# Autodesk Inventor assembly: NSFMKRRA10-131-F3-S5-KA5-A19-KB111.5-B11
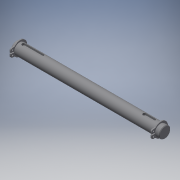
[picture p0: Inventor's stored thumbnail of the model, 180x180]
Saved by Autodesk Inventor 2019 (Build 230136000, 136)
## iProperties
Category: PARTsolutions
Company: MISUMI
Created: 2022-11-16
Part Number: NSFMKRRA10-131-F3-S5-KA5-A19-KB111.5-B11
Catalog Web Link: www.cadenas.de
Description: NSFMKRR, SFMKRR, PSFMKRR, SSFMKRR, NSFHKRR, SFHKRR, PSFHKRR, SSFHKRR, NSFGKRR, SFGKRR, PSFGKRR, SSFGKRR, NSFMKRRA, SFMKRRA, PSFMKRRA, SSFMKRRA, NSFHKRRA, SFHKRRA, PSFHKRRA, SSFHKRRA, NSFGKRRA, SFGKRRA, PSFGKRRA, SSFGKRRA-Rotary Shafts - Retaining Ring Grooves on Both Ends with Keyway -
Vendor: MISUMI
Document SubType Name: Assembly
Designer: psAdmin
Manufacturer: MISUMI
Mass: 10.2368 g
Surface Area: 47.8895 cm^2
Volume: 10.2368 cm^3
Density: 1 g/cm^3
Title: NSFMKRRA10-131-F3-S5-KA5-A19-KB111.5-B11
Author: Cadenas PARTsolutions
Comments: Rotary Shafts - Retaining Ring Grooves on Both Ends with Keyway -
PSOL_IDENT_0: {$CADENAS_DATA/23d-libs/misumi/metric/11_rotary_shafts/psfgkrr_asmtab.prj},644 {VTYP=3D},{STYP=ASSTA
PSOL_IDENT_1: B},{NB=NSFMKRRA10-131-F3-S5-KA5-A19-KB111.5-B11},{LINA=NSFMKRRA10-131-F3-S5-KA5-A19-KB111.5-B11},{NN=
PSOL_IDENT_2: NSFMKRR, SFMKRR, PSFMKRR, SSFMKRR, NSFHKRR, SFHKRR, PSFHKRR, SSFHKRR, NSFGKRR, SFGKRR, PSFGKRR, SSFG
PSOL_IDENT_3: KRR, NSFMKRRA, SFMKRRA, PSFMKRRA, SSFMKRRA, NSFHKRRA, SFHKRRA, PSFHKRRA, SSFHKRRA, NSFGKRRA, SFGKRRA
PSOL_IDENT_4: , PSFGKRRA, SSFGKRRA},{DATE=25.01.2022 23:09:58},{GEOMDATE=05.02.2021 08:16:43},{VERSION=},{LINEID=3
PSOL_IDENT_5: 0},{WBVAR=TS,TYS,MAT,ST,ALT1,L,F,S,NOK,KA,A,KB,B,KC,C,ALT3,FC,GALT3,WFC,J,WALT3,V,ALT4,SFC,SG,AG,ALT
PSOL_IDENT_6: 10,KWC,ALT11,WC,ALT5,UC,ALT7,SC,ALT32,CD},{WBNUMERIC=L,F,S,KA,A,KB,B,KC,C,FC,GALT3,WFC,J,WALT3,V,SFC
PSOL_IDENT_7: ,SG,AG,KWC,WC,UC,SC}  {NB=NSFMKRRA10-131-F3-S5-KA5-A19-KB111.5-B11},{LINA=NSFMKRRA10-131-F3-S5-KA5-A
PSOL_IDENT_8: 19-KB111.5-B11},{KT=DUMMY},{PN=NSFMKRRA10-131-F3-S5-KA5-A19-KB111.5-B11},{TS=A},{TSALG='','Standard'
PSOL_IDENT_9: ,'A','Retaining Ring'},{TYS=M},{TYSALG= 'M','h9 (Cold-drawn)','H','h7 (Ground)','G','g6 (Ground)' },
PSOL_IDENT_10: {MAT=S45C},{MATALG= 'S45C','S45C Equivalent', 'SUS304','304 Stainless Steel' },{ST=},{STALG= '','-','
PSOL_IDENT_11: BO','Black Oxide', 'ENP','Electroless Nickel Plating' },{TYPE=NSFMKRR},{D=10},{ALT1=},{LKCMAX=799.9}
PSOL_IDENT_12: ,{L=131.0},{LALG=[15:800/0.1]},{LMIN=15},{LMAX=800},{F=3.0},{FALG=[3:126/0.1]},{FMIN=3},{FMAX1=122.8
PSOL_IDENT_13: },{FMIN2=6.2},{FMAX2=126},{S=5.0},{SALG=[3:126/0.1]},{SMIN1=3},{SMAX1=121},{SMIN2=6.2},{SMAX2=126},{
PSOL_IDENT_14: DD=9.6},{MM=1.15},{MMALG=1.2},{MMJ=2},{NOK=2},{NOKALG= '1', 'with 1 Key Groove', '2'  , 'with 2 Key
PSOL_IDENT_15: Grooves', '3'  , 'with 3 Key Grooves'},{CIFNOK1=0},{CIFNOK2=3},{CIFNOK3=0},{TOL1=0},{TOL2=3},{TOL3=0
PSOL_IDENT_16: },{BB=3},{TT=1.8},{KA=5.0},{KAALG=[5:116/0.1]},{KAMIN1=0},{KAMIN2=5},{KAMIN3=129.2},{KAMAX1=-1000},{
PSOL_IDENT_17: KAMAX2=116},{KAMAX3=-1000},{A=19.0},{AALG=[3:100/0.1]},{AMIN=3},{AMAX=100},{AMAX1=-1000},{AMAX2=100}
PSOL_IDENT_18: ,{AMAX3=-1000},{KAPN=-KA5-A19},{KB=111.5},{KBALG=[26:121/0.1]},{KBMIN1=26},{KBMIN2=26},{KBMIN3=129.2
PSOL_IDENT_19: },{KBMAX1=-1000},{KBMAX2=121},{KBMAX3=-1000},{B=11.0},{BALG=[3:12.5/0.1]},{BMIN=3},{BMAX=12.5},{BMAX
PSOL_IDENT_20: 1=-1000},{BMAX2=12.5},{BMAX3=-1000},{KBPN=-KB111.5-B11},{KC=0.0},{KCALG=[0]},{KCMIN1=124.5},{KCMIN2=
PSOL_IDENT_21: 124.5},{KCMIN3=129.2},{KCMAX1=-1000},{KCMAX2=-1000},{KCMAX3=-1000},{C=0.0},{CALG=0},{CMIN=3},{CMAX=-
PSOL_IDENT_22: 1000},{CMAX1=-1000},{CMAX2=-1000},{CMAX3=-1000},{CIFKA=5},{CIFKB=3},{CIFKC=3},{KCPN=},{ALT3=},{ALT3A
PSOL_IDENT_23: LG= '', 'w/o Set Screw Flat','FC','with FC (Adds a Set Screw Flat)','WFC','with WFC (Adds Two Set Sc
PSOL_IDENT_24: rew Flats)','FCWFC','with FC + WFC (Adds Three Set Screw Flats)' },{ALT3PN=},{FC=0},{FCALG=[0]},{FCM
PSOL_IDENT_25: IN=0},{FCMAX=130},{GALT3=0},{GALT3ALG=[0]},{GALT3MIN=1},{GALT3MAX=70},{GALT3MAX2=70},{GALT3MAX3=70},
PSOL_IDENT_26: {WFC=0},{WFCALG=[0]},{WFCMIN=0},{WFCMIN2=2},{WFCMAX=127},{WFCMAX2=-3},{WFCMAX3=-4},{J=0},{JALG=[0]},
PSOL_IDENT_27: {JMIN=1},{JMAX=70},{JMAX2=-2},{JMAX3=-5},{WALT3=0},{WALT3ALG=[0]},{WALT3MIN=0},{WALT3MIN2=133},{WALT
PSOL_IDENT_28: 3MAX=128},{WALT3MAX2=128},{V=0},{VALG=[0]},{VMIN=1},{VMAX=70},{VMAX2=70},{CIFFC=0},{ALT4=},{ALT4ALG=
PSOL_IDENT_29: '', 'w/o SFC (2 Set Screw Flats (Angle Specified))', 'SFC'  , 'with SFC (2 Set Screw Flats (Angle S
PSOL_IDENT_30: pecified))'},{ALT4PN=},{SFC=0},{SFCALG=[0]},{SFCMIN=0},{SFCMAX=130},{SG=0},{SGALG=[0]},{SGMIN=1},{SG
PSOL_IDENT_31: MAX=70},{AG=0},{AGALG=[0]},{H=0},{CIFSFC=0},{ALT10=},{ALT10ALG= '','Not applicable' },{KWC=0},{KWCAL
PSOL_IDENT_32: G=[0]},{KWCMIN=1},{KWCMAX=0},{WALT10=8},{ALT10PN=},{ALT11=},{ALT11ALG= '','Not applicable' },{WC=0.0
PSOL_IDENT_33: },{WCALG=[0]},{ALT11PN=},{ALT5=},{ALT5ALG= '', 'w/o UC (Slit Cam Groove)', 'UC', 'with UC (Slit Cam
PSOL_IDENT_34: Groove)'},{ALT5PN=},{UC=0},{UCALG=[0]},{UCMIN=1},{UCMAX=125},{DDALT5=0},{LL1=0},{ALT7=},{ALT7ALG= ''
PSOL_IDENT_35: , 'w/o SC (Wrench Flats)', 'SC', 'with SC (Wrench Flats)'},{ALT7PN=},{SC=0},{SCALG=[0]},{SCMIN=0},{S
PSOL_IDENT_36: CMAX=123},{LL2=0},{LL2ALG=8},{WALT7=0},{CIFSC=0},{ALT32=},{ALT32ALG= '','w/o CD (Changes Part D Cham
PSOL_IDENT_37: fering)','CD','with CD (Changes Part D Chamfering)' },{CD=},{CDALG= '','N/A' },{CD3D=0.5},{ALT32PN=}
PSOL_IDENT_38: ,{CIF323R=0},{CIF323L=0},{CIF324R=0},{CIF324L=0},{CIF3210=0},{CIF32F=0},{CIF32S=0},{ERRORPN=},{ERROR
PSOL_IDENT_39: KGALT3=OK},{ERRORKGALT4=OK},{ERRORKGALT5=OK},{ERRORKGALT7=OK},{ERRORKGALT10=OK},{ERRORRALT3=OK},{ERR
PSOL_IDENT_40: ORRALT4=NG},{ERRORRALT5=NG},{ERRORRALT7=NG},{ERRORRALT10=OK},{ERRORALT34=OK},{ERRORALT35=OK},{ERRORA
PSOL_IDENT_41: LT37=OK},{ERRORALT310=OK},{ERRORALT45=OK},{ERRORALT47=OK},{ERRORALT410=OK},{ERRORALT57=OK},{ERRORALT
PSOL_IDENT_42: 510=OK},{ERRORALT710=OK},{PCUT3D=0},{QCUT3D=0},{TTALT2=1.8},{BBALT2=3},{PPATH=11_components/psfgkrr/
PSOL_IDENT_43: psfgkrr_asmtpl.prj}
NB: NSFMKRRA10-131-F3-S5-KA5-A19-KB111.5-B11
NN: NSFMKRR, SFMKRR, PSFMKRR, SSFMKRR, NSFHKRR, SFHKRR, PSFHKRR, SSFHKRR, NSFGKRR, SFGKRR, PSFGKRR, SSFGKRR, NSFMKRRA, SFMKRRA, PSFMKRRA, SSFMKRRA, NSFHKRRA, SFHKRRA, PSFHKRRA, SSFHKRRA, NSFGKRRA, SFGKRRA, PSFGKRRA, SSFGKRRA
NT: Rotary Shafts - Retaining Ring Grooves on Both Ends with Keyway -
NBSYN: $PN.
LINA: NSFMKRRA10-131-F3-S5-KA5-A19-KB111.5-B11
CATALOG: Misumi
PN: NSFMKRRA10-131-F3-S5-KA5-A19-KB111.5-B11
TS: Retaining Ring
TYS: h9 (Cold-drawn)
MAT: S45C Equivalent
ST: -
D: 10
ALT1: w/o LKC (Changes L Tolerance)
L: 131
F: 3
S: 5
DD: 9.6
MM: 1.15
NOK: with 2 Key Grooves
KA: 5
A: 19
KB: 111.5
B: 11
KC: 0
C: 0
ALT3: w/o Set Screw Flat
FC: 0
GALT3: 0
WFC: 0
J: 0
WALT3: 0
V: 0
ALT4: w/o SFC (2 Set Screw Flats (Angle Specified))
SFC: 0
SG: 0
AG: 0
H: 0
ALT10: Not applicable
KWC: 0
ALT11: Not applicable
WC: 0
ALT5: w/o UC (Slit Cam Groove)
UC: 0
DDALT5: 0
LL1: 0
ALT7: w/o SC (Wrench Flats)
SC: 0
LL2: 0
WALT7: 0
ALT32: w/o CD (Changes Part D Chamfering)
CD: N/A
SUPPLIER: MISUMI
ARTICLENO: NSFMKRRA10-131-F3-S5-KA5-A19-KB111.5-B11
BOMINFO: NSFMKRRA10-131-F3-S5-KA5-A19-KB111.5-B11
CREATOR: CADENAS GmbH
## Documents named in this file (3)
- e:\temp\worker_COMMON_4\temp\tmp_3352_176_HThwi\format_0\NSFMKRRA10-131-F3-S5-KA5-A19-KB111_5-B11.iam
- e:\temp\worker_COMMON_4\temp\tmp_3352_176_HThwi\format_0\NSFMKRRA10-131-F3-S5-KA5-A19-KB111_5-B11_s.ipt
- e:\temp\worker_COMMON_4\temp\tmp_3352_176_HThwi\format_0\STWS10.ipt
## Components (3 placed, 2 different names)
1. NSFMKRRA10-131-F3-S5-KA5-A19-KB111_5-B11_s:1 — to_rring_1_XY@1 <-> 1_XY@2, to_rring_1_Z@1 <-> 1_Z@2, to_rring_1_YZ@1 <-> 1_YZ@2, to_rring_2_XY@1 <-> 1_XY@3, to_rring_2_Z@1 <-> 1_Z@3, to_rring_2_YZ@1 <-> 1_YZ@3
2. STWS10:1 — to_rring_1_XY@1 <-> 1_XY@2, to_rring_1_Z@1 <-> 1_Z@2, to_rring_1_YZ@1 <-> 1_YZ@2
3. STWS10:2 — to_rring_2_XY@1 <-> 1_XY@3, to_rring_2_Z@1 <-> 1_Z@3, to_rring_2_YZ@1 <-> 1_YZ@3
## Relationships (6: Mate 4, Angle 2)
- to_rring_1_XY@1 <-> 1_XY@2 [Mate]: NSFMKRRA10-131-F3-S5-KA5-A19-KB111_5-B11_s:1 ↔ STWS10:1
- to_rring_1_Z@1 <-> 1_Z@2 [Mate]: NSFMKRRA10-131-F3-S5-KA5-A19-KB111_5-B11_s:1 ↔ STWS10:1
- to_rring_1_YZ@1 <-> 1_YZ@2 [Angle] (180 deg): NSFMKRRA10-131-F3-S5-KA5-A19-KB111_5-B11_s:1 ↔ STWS10:1
- to_rring_2_XY@1 <-> 1_XY@3 [Mate]: NSFMKRRA10-131-F3-S5-KA5-A19-KB111_5-B11_s:1 ↔ STWS10:2
- to_rring_2_Z@1 <-> 1_Z@3 [Mate]: NSFMKRRA10-131-F3-S5-KA5-A19-KB111_5-B11_s:1 ↔ STWS10:2
- to_rring_2_YZ@1 <-> 1_YZ@3 [Angle] (180 deg): NSFMKRRA10-131-F3-S5-KA5-A19-KB111_5-B11_s:1 ↔ STWS10:2
